# Autodesk Inventor assembly: PitchMotor
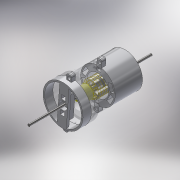
[picture p0: Inventor's stored thumbnail of the model, 180x180]
Saved by Autodesk Inventor 2018 (Build 220112000, 112)
## iProperties
Created: 2018-02-06
Part Number: PitchMotor
Document SubType Name: Assembly
Designer: mansu
Author: mansu
Sending System: SolidWorks 2017
Last Author: leoli
Last Saved: 2018-03-25
## Documents named in this file (7)
- F:\OneDrive\Documents\2018 UBC\ELEC 391\Controller\cad\PitchMotor.iam
- F:\OneDrive\Documents\2018 UBC\ELEC 391\Motor\SolidWorks\Pitch\pitch_RotorCore.ipt
- F:\OneDrive\Documents\2018 UBC\ELEC 391\Motor\SolidWorks\Pitch\pitch_shaft.ipt
- F:\OneDrive\Documents\2018 UBC\ELEC 391\Motor\SolidWorks\Pitch\pitch_StatorShell_v5.ipt
- F:\OneDrive\Documents\2018 UBC\ELEC 391\Motor\SolidWorks\Pitch\pitch_StatorShell_v5_attachment.ipt
- F:\OneDrive\Documents\2018 UBC\ELEC 391\Motor\SolidWorks\Pitch\pitch_StatorShell_v1_Top_Flashlight_attachment.ipt
- F:\OneDrive\Documents\2018 UBC\ELEC 391\Motor\SolidWorks\Pitch\pitch_commutator_attachment1.ipt
## Components (6 placed, 6 different names)
1. pitch_RotorCore:1 — Mate:1, Mate:2, Mate:6, Mate:7
2. pitch_shaft:1 — Mate:3, Mate:5
3. pitch_StatorShell_v5:1 — Mate:1, Mate:6, Mate:8, Mate:9
4. pitch_StatorShell_v5_attachment:1 — Mate:4, Mate:8, Mate:9, Mate:10, Mate:11
5. pitch_StatorShell_v1_Top_Flashlight_attachment:1 — Mate:5, Mate:10, Mate:11
6. pitch_commutator_attachment1:1 — Mate:2, Mate:3, Mate:4, Mate:7
## Relationships (11: Mate 11)
- Mate:1: pitch_RotorCore:1 ↔ pitch_StatorShell_v5:1
- Mate:2: pitch_RotorCore:1 ↔ pitch_commutator_attachment1:1
- Mate:3: pitch_shaft:1 ↔ pitch_commutator_attachment1:1
- Mate:4: pitch_StatorShell_v5_attachment:1 ↔ pitch_commutator_attachment1:1
- Mate:5: pitch_shaft:1 ↔ pitch_StatorShell_v1_Top_Flashlight_attachment:1
- Mate:6 (5 mm): pitch_RotorCore:1 ↔ pitch_StatorShell_v5:1
- Mate:7 (5 mm): pitch_RotorCore:1 ↔ pitch_commutator_attachment1:1
- Mate:8: pitch_StatorShell_v5:1 ↔ pitch_StatorShell_v5_attachment:1
- Mate:9 (0.1 mm): pitch_StatorShell_v5:1 ↔ pitch_StatorShell_v5_attachment:1
- Mate:10: pitch_StatorShell_v5_attachment:1 ↔ pitch_StatorShell_v1_Top_Flashlight_attachment:1
- Mate:11 (0.1 mm): pitch_StatorShell_v5_attachment:1 ↔ pitch_StatorShell_v1_Top_Flashlight_attachment:1
